# Autodesk Inventor assembly: PlanetaryGearConstruction
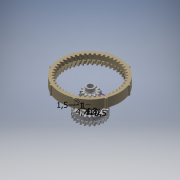
[picture p0: Inventor's stored thumbnail of the model, 180x180]
Saved by Autodesk Inventor 2019.1 (Build 231200000, 200)
## iProperties
Created: 2019-01-01
Part Number: PlanetaryGearConstruction
Material: Generisch
Document SubType Name: Assembly
Designer: JochenAlt
Author: JochenAlt
## Documents named in this file (3)
- D:\Projects\Ondine\CAD\PlanetaryGear2\PlanetaryGearConstruction.iam
- D:\Projects\Ondine\CAD\PlanetaryGear2\PlanetaryGearConstruction\Stirnräder1.iam
- D:\Projects\Ondine\CAD\PlanetaryGear2\PlanetaryGearConstruction\Stirnräder2.iam
## Components (2 placed, 1 different names)
1. Stirnräder:1 [sub-assembly] — Passend:9, Passend:19, Passend:20, Passend:21
2. Stirnräder:2 [sub-assembly] — Passend:9, Passend:21
## Relationships (4: Mate 4)
- Passend:9 [Mate]: Stirnräder:1 ↔ Stirnräder:2
- Passend:19 [Mate]: Stirnräder:1
- Passend:20 [Mate]: Stirnräder:1
- Passend:21 [Mate]: Stirnräder:1 ↔ Stirnräder:2
